# Autodesk Inventor assembly: blokken
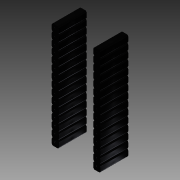
[picture p0: Inventor's stored thumbnail of the model, 180x180]
Saved by Autodesk Inventor 2015 (Build 190159000, 159)
## iProperties
Created: 2015-12-04
Part Number: blokken
Document SubType Name: Assembly
Designer: david
Author: david
## Documents named in this file (2)
- Z:\gip\generatie 6\frame\bak\electronica\printplaat\blokken.iam
- Z:\gip\generatie 6\frame\bak\electronica\printplaat\block.ipt
## Components (30 placed, 1 different names)
1. block:1
2. block:2
3. block:3
4. block:4
5. block:5
6. block:6
7. block:7
8. block:8
9. block:9
10. block:10
11. block:11
12. block:12
13. block:13
14. block:14
15. block:15
16. block:16
17. block:17
18. block:18
19. block:19
20. block:20
21. block:21
22. block:22
23. block:23
24. block:24
25. block:25
26. block:26
27. block:27
28. block:28
29. block:29
30. block:30
## Component patterns: (30 elements, first: block:1)
